# Autodesk Inventor assembly: Project
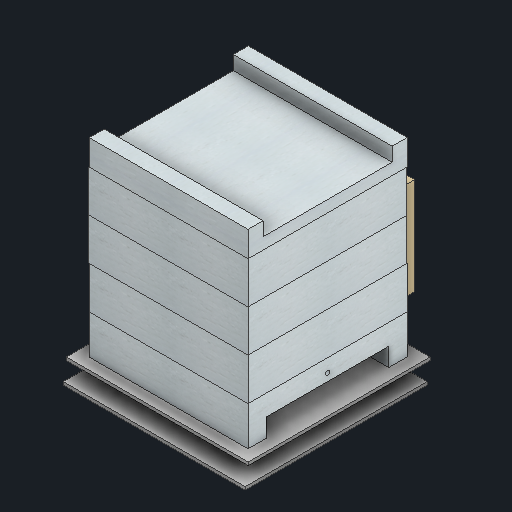
[picture p0: Inventor's stored thumbnail of the model, 512x512]
Saved by Autodesk Inventor 2027 (Build 310192060, 192F)
## iProperties
Created: 2026-10-02
Part Number: Project
Document SubType Name: Assembly
Designer: notra
Author: notra
## Documents named in this file (4)
- C:\Users\notra\Desktop\BeeBox\3dFiles\Project.iam
- C:\Users\notra\Desktop\BeeBox\3dFiles\Colmeia.iam
- C:\Users\notra\Desktop\BeeBox\3dFiles\Beebox_ass.iam
- C:\Users\notra\Documents\Pedro\SBESC\Model3D\LoadCellAssembly.iam
## Components (3 placed, 3 different names)
1. Colmeia:1 [sub-assembly] — Mate:1, Flush:1, Flush:2, Mate:2, Rigid:1
2. Beebox_ass:1 [sub-assembly] — Mate:1, Flush:1, Flush:2
3. LoadCellAssembly:1 [sub-assembly] — Mate:2, Rigid:1
## Relationships (5: Mate 2, Flush 2, WeldJoint 1)
- Mate:1: Colmeia:1 ↔ Beebox_ass:1
- Flush:1 (50 mm): Colmeia:1 ↔ Beebox_ass:1
- Flush:2 (37 mm): Colmeia:1 ↔ Beebox_ass:1
- Mate:2: Colmeia:1 ↔ LoadCellAssembly:1
- Rigid:1 [WeldJoint] (30.4 mm): Colmeia:1 ↔ LoadCellAssembly:1
